# Autodesk Inventor assembly: FingertipTestAssembly
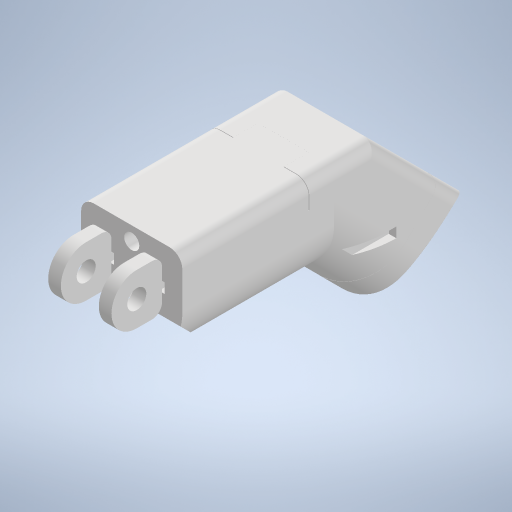
[picture p0: Inventor's stored thumbnail of the model, 512x512]
Saved by Autodesk Inventor 2023 (Build 270158000, 158)
## iProperties
Created: 2023-04-11
Part Number: FingertipTestAssembly
Document SubType Name: Assembly
Designer: 1roweste
Author: 1roweste
## Documents named in this file (5)
- G:\MyPortfolio\Grade 12 Robotics\Robotic Arm project\FingertipTestAssembly.iam
- G:\MyPortfolio\Grade 12 Robotics\Robotic Arm project\Fingertip Midpart.ipt
- G:\MyPortfolio\Grade 12 Robotics\Robotic Arm project\Fingertip End.ipt
- G:\MyPortfolio\Grade 12 Robotics\Robotic Arm project\FingerTip Hardtip.ipt
- G:\MyPortfolio\Grade 12 Robotics\Robotic Arm project\Knuckle Attachment DirectInsert.ipt
## Components (5 placed, 4 different names)
1. Fingertip Midpart:1 — Mate:1, Flush:1, Flush:2, Mate:2, Mate:5, Mate:6, Mate:7, Mate:8, Mate:9, Mate:10
2. Fingertip End:1 — Mate:1, Flush:1, Flush:2, Mate:2, Mate:3, Flush:3, Mate:4
3. FingerTip Hardtip:1 — Mate:3, Flush:3, Mate:4
4. Knuckle Attachment DirectInsert:1 — Mate:5, Mate:6, Mate:7
5. Knuckle Attachment DirectInsert:2 — Mate:8, Mate:9, Mate:10
## Relationships (13: Mate 10, Flush 3)
- Mate:1: Fingertip Midpart:1 ↔ Fingertip End:1
- Flush:1: Fingertip Midpart:1 ↔ Fingertip End:1
- Flush:2: Fingertip Midpart:1 ↔ Fingertip End:1
- Mate:2: Fingertip Midpart:1 ↔ Fingertip End:1
- Mate:3: Fingertip End:1 ↔ FingerTip Hardtip:1
- Flush:3: Fingertip End:1 ↔ FingerTip Hardtip:1
- Mate:4: Fingertip End:1 ↔ FingerTip Hardtip:1
- Mate:5: Fingertip Midpart:1 ↔ Knuckle Attachment DirectInsert:1
- Mate:6: Fingertip Midpart:1 ↔ Knuckle Attachment DirectInsert:1
- Mate:7: Fingertip Midpart:1 ↔ Knuckle Attachment DirectInsert:1
- Mate:8: Fingertip Midpart:1 ↔ Knuckle Attachment DirectInsert:2
- Mate:9: Fingertip Midpart:1 ↔ Knuckle Attachment DirectInsert:2
- Mate:10: Fingertip Midpart:1 ↔ Knuckle Attachment DirectInsert:2
